# Autodesk Inventor assembly: printer
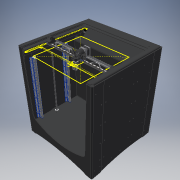
[picture p0: Inventor's stored thumbnail of the model, 180x180]
Saved by Autodesk Inventor 2016 (Build 200138000, 138)
## iProperties
Created: 2016-06-10
Part Number: printer
Document SubType Name: Assembly
Designer: brent
Author: brent
## Documents named in this file (6)
- C:\Users\brent\OneDrive\personal\printer_cad\printer.iam
- C:\Users\brent\OneDrive\personal\printer_cad\frame.ipt
- C:\Users\brent\OneDrive\personal\printer_cad\x_gantry.iam
- C:\Users\brent\OneDrive\personal\printer_cad\offtheshelf\linear_stepper_350mm.ipt
- C:\Users\brent\OneDrive\personal\printer_cad\offtheshelf\sbr12_350mm.ipt
- C:\Users\brent\OneDrive\personal\printer_cad\offtheshelf\nema17_40mm.ipt
## Components (10 placed, 5 different names)
1. frame:1 — Mate:2, Mate:3, Mate:4, Mate:5, Mate:6, Mate:7, Mate:8, Mate:9, Mate:10, Mate:11, Mate:12, Mate:13, Mate:14, Mate:15, Mate:16, Mate:17, Mate:18, Mate:19, Mate:20, Mate:21, Mate:22, Mate:23
2. x_gantry:1 [sub-assembly] — Mate:2, Mate:3
3. linear_stepper_350mm:1 — Mate:4, Mate:7
4. linear_stepper_350mm:2 — Mate:5, Mate:6
5. sbr12_350mm:1 — Mate:8, Mate:9, Mate:10
6. sbr12_350mm:2 — Mate:14, Mate:15, Mate:16
7. sbr12_350mm:3 — Mate:17, Mate:18, Mate:19
8. sbr12_350mm:4 — Mate:11, Mate:12, Mate:13
9. nema17_40mm:1 — Mate:22, Mate:23
10. nema17_40mm:2 — Mate:20, Mate:21
## Relationships (22: Mate 22)
- Mate:2 (5 mm): frame:1 ↔ x_gantry:1
- Mate:3 (6.5 mm): frame:1 ↔ x_gantry:1
- Mate:4: frame:1 ↔ linear_stepper_350mm:1
- Mate:5: frame:1 ↔ linear_stepper_350mm:2
- Mate:6: frame:1 ↔ linear_stepper_350mm:2
- Mate:7: frame:1 ↔ linear_stepper_350mm:1
- Mate:8: frame:1 ↔ sbr12_350mm:1
- Mate:9: frame:1 ↔ sbr12_350mm:1
- Mate:10: frame:1 ↔ sbr12_350mm:1
- Mate:11: frame:1 ↔ sbr12_350mm:4
- Mate:12: frame:1 ↔ sbr12_350mm:4
- Mate:13: frame:1 ↔ sbr12_350mm:4
- Mate:14: frame:1 ↔ sbr12_350mm:2
- Mate:15: frame:1 ↔ sbr12_350mm:2
- Mate:16: frame:1 ↔ sbr12_350mm:2
- Mate:17: frame:1 ↔ sbr12_350mm:3
- Mate:18: frame:1 ↔ sbr12_350mm:3
- Mate:19: frame:1 ↔ sbr12_350mm:3
- Mate:20: frame:1 ↔ nema17_40mm:2
- Mate:21: frame:1 ↔ nema17_40mm:2
- Mate:22: frame:1 ↔ nema17_40mm:1
- Mate:23: frame:1 ↔ nema17_40mm:1
